# Autodesk Inventor assembly: Anderson_w-hook
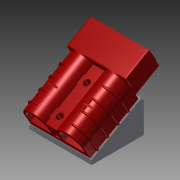
[picture p0: Inventor's stored thumbnail of the model, 180x180]
Saved by Autodesk Inventor 2015 (Build 190159000, 159)
## iProperties
Created: 2015-02-09
Part Number: Anderson_w-hook
Document SubType Name: Assembly
Designer: whitaus15
Author: whitaus15
## Documents named in this file (3)
- \\lhssvr02\Homedirs\Robotics Club\CAD Model 2015\Box Beam Drive Base\Newest\Anderson_w-hook.iam
- \\lhssvr02\Homedirs\Robotics Club\CAD Model 2015\Parts Folder\Electrical\Anderson SB50.ipt
- \\lhssvr02\Homedirs\Robotics Club\CAD Model 2015\Box Beam Drive Base\Newest\Anderson Holder.ipt
## Components (2 placed, 2 different names)
1. Anderson SB50:1 — Mate:3, Mate:4, Tangent:1
2. Anderson Holder:1 — Mate:3, Mate:4, Tangent:1
## Relationships (3: Mate 2, Tangent 1)
- Mate:3: Anderson SB50:1 ↔ Anderson Holder:1
- Mate:4: Anderson SB50:1 ↔ Anderson Holder:1
- Tangent:1: Anderson SB50:1 ↔ Anderson Holder:1
